# Autodesk Inventor assembly: Horizntal Leg Test
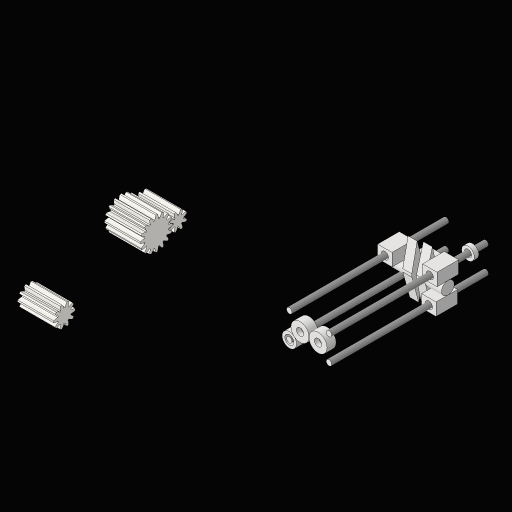
[picture p0: Inventor's stored thumbnail of the model, 512x512]
Saved by Autodesk Inventor 2023.2 (Build 272271030, 271C)
## iProperties
Created: 2023-11-10
Part Number: Horizntal Leg Test
Document SubType Name: Assembly
Designer: robpl
Author: robpl
## Documents named in this file (12)
- C:\Users\robpl\OneDrive\Documents\Arduino\Onslaught\CAD\Horizontal Leg Test\Horizntal Leg Test.iam
- C:\Users\robpl\OneDrive\Documents\Arduino\Onslaught\CAD\Frame Test\M4 Leg Throd.ipt
- C:\Users\robpl\OneDrive\Documents\Arduino\Onslaught\CAD\Horizontal Leg Test\Leg.ipt
- C:\Users\robpl\OneDrive\Documents\Arduino\Onslaught\CAD\Horizontal Leg Test\Rack.ipt
- C:\Users\robpl\OneDrive\Documents\Arduino\Onslaught\CAD\Horizontal Leg Test\N20 DC MOTOR Gearbox\N20 DC MOTOR Gearbox.ipt
- C:\Users\robpl\OneDrive\Documents\Arduino\Onslaught\CAD\Horizontal Leg Test\Throd Drive Gear.ipt
- C:\Users\robpl\OneDrive\Documents\Arduino\Onslaught\CAD\Horizontal Leg Test\Motor Drive Gear.ipt
- C:\Users\robpl\OneDrive\Documents\Arduino\Onslaught\CAD\Horizontal Leg Test\4x7x2.5mm Bearing.ipt
- C:\Users\robpl\OneDrive\Documents\Arduino\Onslaught\CAD\Horizontal Leg Test\PTA6043-2015DPA103--3DModel-STEP-269445\PTA6043-2015DPA103--3DModel-STEP-269445.ipt
- C:\Users\robpl\OneDrive\Documents\Arduino\Onslaught\CAD\Horizontal Leg Test\Idler Gear.ipt
- C:\Users\robpl\OneDrive\Documents\Arduino\Onslaught\CAD\Horizontal Leg Test\Horizntal Leg Test\Design Accelerator\Spur Gears2.iam
- C:\Users\robpl\OneDrive\Documents\Arduino\Onslaught\CAD\Horizontal Leg Test\Horizntal Leg Test\Design Accelerator\Spur Gears3.iam
## Components (25 placed, 10 different names)
1. N20 DC MOTOR Gearbox:2 — Mate:12, Flush:15, Flush:17, Flush:30
2. M4 Leg Throd:1 — Flush:1, Mate:7, Mate:9, Flush:12, Flush:27
3. M4 Leg Throd:2 — Flush:1, Mate:6, Mate:11, Flush:13, Mate:14
4. Leg:1 — Tangent:1, Tangent:2, Flush:31, Mate:21
5. Rack:1 — Mate:7, Tangent:2, Flush:31, Flush:26, Flush:34
6. Rack:2 — Mate:6, Tangent:1, Angle:1, Flush:34
7. N20 DC MOTOR Gearbox:1 — Mate:10, Flush:17, Flush:18
8. Throd Drive Gear:1 — Mate:9, Tangent:3, Flush:12, Flush:19, Tangent:8, Flush:36
9. Motor Drive Gear:1 — Mate:10, Tangent:3, Flush:18, Flush:19, Mate:13
10. Motor Drive Gear:2 — Mate:12, Tangent:4, Flush:14, Flush:15, Mate:13
11. Throd Drive Gear:2 — Mate:11, Flush:13, Tangent:4, Flush:14
12. 4x7x2.5mm Bearing:1 — Mate:14
13. PTA6043-2015DPA103--3DModel-STEP-269445:1 — Flush:21, Flush:28, Mate:22, Flush:29, Mate:23
14. PTA6043-2015DPA103--3DModel-STEP-269445:2 — Flush:21, Flush:28, Mate:22, Flush:30
15. M4 Leg Throd:3 — Mate:24
16. M4 Leg Throd:4 — Flush:27, Mate:25
17. Leg:2 — Flush:32, Mate:21
18. Rack:3 — Flush:32, Flush:33
19. Rack:4 — Flush:26, Flush:29, Flush:33, Mate:23
20. Throd Drive Gear:3 — Mate:25, Flush:35, Tangent:7
21. Throd Drive Gear:4 — Mate:24
22. Idler Gear:1 — Flush:35, Tangent:7, Tangent:9
23. Idler Gear:2 — Tangent:8, Flush:36, Tangent:9
24. Spur Gears:1 [sub-assembly]
25. Spur Gears:2 [sub-assembly]
## Relationships (48: Flush 23, Mate 15, Tangent 9, Angle 1)
- Flush:1: M4 Leg Throd:1 ↔ M4 Leg Throd:2
- Mate:6: M4 Leg Throd:2 ↔ Rack:2
- Mate:7: M4 Leg Throd:1 ↔ Rack:1
- Tangent:1: Leg:1 ↔ Rack:2
- Tangent:2: Leg:1 ↔ Rack:1
- Flush:31: Leg:1 ↔ Rack:1
- Mate:9: M4 Leg Throd:1 ↔ Throd Drive Gear:1
- Mate:10: N20 DC MOTOR Gearbox:1 ↔ Motor Drive Gear:1
- Tangent:3: Throd Drive Gear:1 ↔ Motor Drive Gear:1
- Flush:12: M4 Leg Throd:1 ↔ Throd Drive Gear:1
- Mate:11: M4 Leg Throd:2 ↔ Throd Drive Gear:2
- Flush:13: M4 Leg Throd:2 ↔ Throd Drive Gear:2
- Mate:12: N20 DC MOTOR Gearbox:2 ↔ Motor Drive Gear:2
- Tangent:4: Motor Drive Gear:2 ↔ Throd Drive Gear:2
- Flush:14: Motor Drive Gear:2 ↔ Throd Drive Gear:2
- Flush:15: N20 DC MOTOR Gearbox:2 ↔ Motor Drive Gear:2
- Angle:1 (90 deg): Rack:2
- Flush:17: N20 DC MOTOR Gearbox:2 ↔ N20 DC MOTOR Gearbox:1
- Flush:18: N20 DC MOTOR Gearbox:1 ↔ Motor Drive Gear:1
- Flush:19: Throd Drive Gear:1 ↔ Motor Drive Gear:1
- Mate:13: Motor Drive Gear:1 ↔ Motor Drive Gear:2
- Mate:14: M4 Leg Throd:2 ↔ 4x7x2.5mm Bearing:1
- Flush:21: PTA6043-2015DPA103--3DModel-STEP-269445:1 ↔ PTA6043-2015DPA103--3DModel-STEP-269445:2
- [Flush]: M4 Leg Throd:3 ↔ M4 Leg Throd:4
- [Mate]: M4 Leg Throd:4 ↔ Rack:4
- [Mate]: M4 Leg Throd:3 ↔ Rack:3
- [Tangent]: Leg:2 ↔ Rack:4
- [Tangent]: Leg:2 ↔ Rack:3
- Flush:32: Leg:2 ↔ Rack:3
- [Flush]: M4 Leg Throd:3 ↔ Throd Drive Gear:3
- [Flush]: M4 Leg Throd:4 ↔ Throd Drive Gear:4
- Flush:26: Rack:1 ↔ Rack:4
- Flush:27: M4 Leg Throd:1 ↔ M4 Leg Throd:4
- Mate:21 (2 mm): Leg:1 ↔ Leg:2
- Flush:28: PTA6043-2015DPA103--3DModel-STEP-269445:1 ↔ PTA6043-2015DPA103--3DModel-STEP-269445:2
- Mate:22 (1 mm): PTA6043-2015DPA103--3DModel-STEP-269445:1 ↔ PTA6043-2015DPA103--3DModel-STEP-269445:2
- Flush:29 (3.4 mm): PTA6043-2015DPA103--3DModel-STEP-269445:1 ↔ Rack:4
- Flush:30: N20 DC MOTOR Gearbox:2 ↔ PTA6043-2015DPA103--3DModel-STEP-269445:2
- Flush:33: Rack:3 ↔ Rack:4
- Flush:34: Rack:1 ↔ Rack:2
- Mate:23: PTA6043-2015DPA103--3DModel-STEP-269445:1 ↔ Rack:4
- Mate:24: M4 Leg Throd:3 ↔ Throd Drive Gear:4
- Mate:25: M4 Leg Throd:4 ↔ Throd Drive Gear:3
- Flush:35: Throd Drive Gear:3 ↔ Idler Gear:1
- Tangent:7: Throd Drive Gear:3 ↔ Idler Gear:1
- Tangent:8: Throd Drive Gear:1 ↔ Idler Gear:2
- Flush:36: Throd Drive Gear:1 ↔ Idler Gear:2
- Tangent:9: Idler Gear:1 ↔ Idler Gear:2
## Named parameters: d45_d9 = 0 mm, d46_d14 = 0 mm, d47_d15 = 0 mm, d48_d16 = 0 mm, d49_d17 = 0 mm, d51_d0 = 0 mm, d53_d23 = 0 mm, d55_d25 = 0 mm
